# Autodesk Inventor assembly: Pre-roller
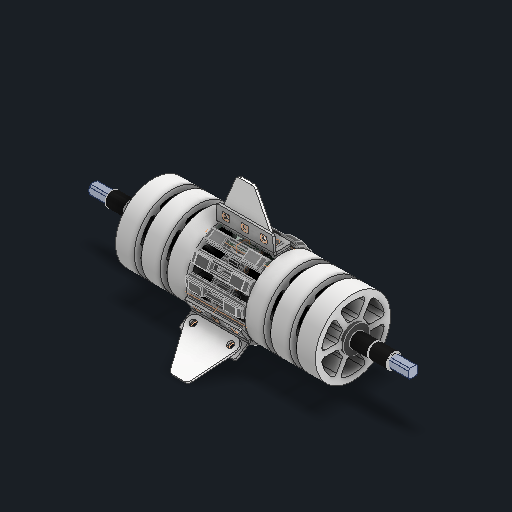
[picture p0: Inventor's stored thumbnail of the model, 512x512]
Saved by Autodesk Inventor 2025.1 (Build 291241000, 241)
## iProperties
Created: 2024-10-21
Part Number: Pre-roller
Document SubType Name: Assembly
Designer: averey
Author: averey
## Documents named in this file (10)
- C:\Users\avere\VEX\High Stakes\CAD\V3\Intake\Floating Stage\Pre-roller.iam
- C:\Users\avere\VEX\High Stakes\CAD\ROBOPROS-CAD-Inventor\Motion\Shaft HS\Shaft HS\Shaft HS 8.5 in.ipt
- C:\Users\avere\VEX\High Stakes\CAD\ROBOPROS-CAD-Inventor\Motion\Shaft HS\Shaft HS.ipt
- C:\Users\avere\VEX\High Stakes\CAD\ROBOPROS-CAD-Inventor\Quick Assemblies\2.000 30A .500 With Adapters.iam
- C:\Users\avere\VEX\High Stakes\CAD\ROBOPROS-CAD-Inventor\Motion\Shaft HS\HS Spacer\HSpacer .5000.ipt
- C:\Users\avere\VEX\High Stakes\CAD\ROBOPROS-CAD-Inventor\Motion\Shaft HS\HS Spacer.ipt
- C:\Users\avere\VEX\High Stakes\CAD\ROBOPROS-CAD-Inventor\Motion\Sprockets\9P Sprocket\9P 12T Sprocket, No Insert.iam
- C:\Users\avere\VEX\High Stakes\CAD\ROBOPROS-CAD-Inventor\Motion\Sprockets\9P Sprocket.iam
- C:\Users\avere\VEX\High Stakes\CAD\V3\Intake\Floating Stage\Flap.iam
- C:\Users\avere\VEX\High Stakes\CAD\ROBOPROS-CAD-Inventor\Motion\Chain 9P\Tank Tread Traction Link.ipt
## Components (27 placed, 6 different names)
1. Shaft HS 8.5 in:1 — Flush:1, Mate:1, Mate:2, Insert:3, Flush:2
2. 2.000 30A .500 With Adapters:1 [sub-assembly] — Insert:1, Mate:3, Insert:8
3. 2.000 30A .500 With Adapters:2 [sub-assembly] — Insert:1, Insert:3, Insert:5
4. 2.000 30A .500 With Adapters:3 [sub-assembly] — Insert:9
5. 2.000 30A .500 With Adapters:4 [sub-assembly] — Mate:3, Flush:2, Insert:7
6. HSpacer .5000:1 — Insert:4, Insert:5
7. HSpacer .5000:2 — Insert:4
8. HSpacer .5000:3
9. HSpacer .5000:4 — Insert:7
10. 2.000 30A .500 With Adapters:5 [sub-assembly] — Insert:8
11. 2.000 30A .500 With Adapters:6 [sub-assembly] — Insert:9, Insert:10
12. 9P 12T Sprocket, No Insert:1 [sub-assembly] — Insert:10, Mate:4, Mate:5, Mate:6
13. Tank Tread Traction Link:1 — Mate:4, Mate:5, Mate:6
14. Tank Tread Traction Link:2
15. Tank Tread Traction Link:3
16. Tank Tread Traction Link:4 — Insert:11
17. Tank Tread Traction Link:5 — Mate:7
18. Tank Tread Traction Link:6
19. Tank Tread Traction Link:7
20. Tank Tread Traction Link:8
21. Tank Tread Traction Link:9
22. Tank Tread Traction Link:10
23. Tank Tread Traction Link:11
24. Tank Tread Traction Link:12
25. Flap:1 [sub-assembly] — Insert:11, Mate:7
26. Flap:2 [sub-assembly]
27. Flap:3 [sub-assembly]
## Component patterns: (12 elements, first: Tank Tread Traction Link:1), (3 elements, first: Flap:1)
## Relationships (20: Insert 11, Mate 7, Flush 2)
- Flush:1 (-107.95 mm): Shaft HS 8.5 in:1
- Mate:1: Shaft HS 8.5 in:1
- Mate:2: Shaft HS 8.5 in:1
- Insert:1: 2.000 30A .500 With Adapters:1 ↔ 2.000 30A .500 With Adapters:2
- [Insert]: 2.000 30A .500 With Adapters:3 ↔ 2.000 30A .500 With Adapters:4
- Insert:3 (38.1 mm): Shaft HS 8.5 in:1 ↔ 2.000 30A .500 With Adapters:2
- Mate:3: 2.000 30A .500 With Adapters:1 ↔ 2.000 30A .500 With Adapters:4
- Flush:2 (38.1 mm): Shaft HS 8.5 in:1 ↔ 2.000 30A .500 With Adapters:4
- Insert:4: HSpacer .5000:1 ↔ HSpacer .5000:2
- Insert:5: 2.000 30A .500 With Adapters:2 ↔ HSpacer .5000:1
- [Insert]: HSpacer .5000:3 ↔ HSpacer .5000:4
- Insert:7: 2.000 30A .500 With Adapters:4 ↔ HSpacer .5000:4
- Insert:8: 2.000 30A .500 With Adapters:1 ↔ 2.000 30A .500 With Adapters:5
- Insert:9: 2.000 30A .500 With Adapters:3 ↔ 2.000 30A .500 With Adapters:6
- Insert:10 (11.18 mm): 2.000 30A .500 With Adapters:6 ↔ 9P 12T Sprocket, No Insert:1
- Mate:4: 9P 12T Sprocket, No Insert:1 ↔ Tank Tread Traction Link:1
- Mate:5: 9P 12T Sprocket, No Insert:1 ↔ Tank Tread Traction Link:1
- Mate:6 (0.3969 mm): 9P 12T Sprocket, No Insert:1 ↔ Tank Tread Traction Link:1
- Insert:11: Tank Tread Traction Link:4 ↔ Flap:1
- Mate:7: Tank Tread Traction Link:5 ↔ Flap:1
## Named parameters: d4_d3 = 0 mm, d10_d8 = 0 mm
